# Autodesk Inventor assembly: Samenstel draaischijf apparte delen
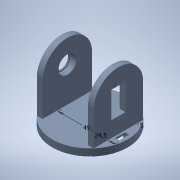
[picture p0: Inventor's stored thumbnail of the model, 180x180]
Saved by Autodesk Inventor 2021 (Build 250183000, 183)
## iProperties
Manager: Pierloot J.
Company: Emmaüs Bovenbouw Aalter
Created: 2021-03-04
Part Number: Samenstel draaischijf apparte delen
Catalog Web Link: http://emmausbovenbouw.op-weg.be/
Vendor: Emmaüs Bovenbouw Aalter
Document SubType Name: Assembly
Designer: iskhak.tchuytiyev
Engineer: Declercq St.
Authority: Declercq St.
Title: Algemene Projecttitel
Author: iskhak.tchuytiyev
## Documents named in this file (4)
- C:\Users\iskhak.tchuytiyev\OneDrive - Emmaus Aalter Secundaire School\Documenten\School\GIP\GIP Inventor\Waterkanon\Samenstel draaischijf apparte delen.iam
- C:\Users\iskhak.tchuytiyev\OneDrive - Emmaus Aalter Secundaire School\Documenten\School\GIP\GIP Inventor\Waterkanon\Draaischijf wand links.ipt
- C:\Users\iskhak.tchuytiyev\OneDrive - Emmaus Aalter Secundaire School\Documenten\School\GIP\GIP Inventor\Waterkanon\Draaischijf wand rechts.ipt
- C:\Users\iskhak.tchuytiyev\OneDrive - Emmaus Aalter Secundaire School\Documenten\School\GIP\GIP Inventor\Waterkanon\Draaischijf wanden draaischijf appart.ipt
## Components (3 placed, 3 different names)
1. Draaischijf wand links:1 — Mate:2, Mate:3, Mate:4
2. Draaischijf wand rechts:1 — Mate:1, Mate:5, Mate:6
3. Draaischijf wanden draaischijf appart:1 — Mate:1, Mate:2, Mate:3, Mate:4, Mate:5, Mate:6
## Relationships (6: Mate 6)
- Mate:1: Draaischijf wand rechts:1 ↔ Draaischijf wanden draaischijf appart:1
- Mate:2: Draaischijf wand links:1 ↔ Draaischijf wanden draaischijf appart:1
- Mate:3: Draaischijf wand links:1 ↔ Draaischijf wanden draaischijf appart:1
- Mate:4: Draaischijf wand links:1 ↔ Draaischijf wanden draaischijf appart:1
- Mate:5: Draaischijf wand rechts:1 ↔ Draaischijf wanden draaischijf appart:1
- Mate:6: Draaischijf wand rechts:1 ↔ Draaischijf wanden draaischijf appart:1
